# Autodesk Inventor assembly: 4thRhinoRobot
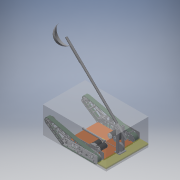
[picture p0: Inventor's stored thumbnail of the model, 180x180]
Saved by Autodesk Inventor 2016 SP1 (Build 200210100, 210)
## iProperties
Created: 2015-12-30
Part Number: 4thRhinoRobot
Document SubType Name: Assembly
Designer: steele
Mass: 23511.9 g
Surface Area: 38256.8 cm^2
Volume: 14882.3 cm^3
Density: 1.57986 g/cm^3
Author: steele
## Documents named in this file (15)
- C:\snobotics\CAD-Development\robSteele\SnoBotics2016\4thCutRhinoRobot\4thRhinoRobot.iam
- C:\snobotics\CAD-Development\robSteele\SnoBotics2016\RhinoTrackDrive\am-3322+RhinoTrackDriveModule.iam
- C:\snobotics\CAD-Development\robSteele\SnoBotics2016\FirstCutRhinoRobot\BasePlate.ipt
- C:\snobotics\CAD-Development\robSteele\SnoBotics2016\RhinoTrackDrive\am-3322+RhinoTrackDriveModule_MIR.iam
- C:\snobotics\autodesk\2015\FRC_KOP_2015\Motors\MOT_CIM-Motor_217-2000.iam
- C:\snobotics\CAD-Development\robSteele\SnoBotics2016\2ndCutAtCatapultRobot\catapultArmSupportStructure.ipt
- C:\snobotics\CAD-Development\robSteele\SnoBotics2016\FirstCutCatapult\CatapultAxel.ipt
- C:\snobotics\CAD-Development\robSteele\SnoBotics2016\2ndCutAtCatapultRobot\6498K330.ipt
- C:\snobotics\CAD-MfgResources\McMaster-Carr\Air Cylinder\Universal Mount\Single Acting Spring Return\3_4 bore 6 stroke\6498K045.ipt
- C:\snobotics\CAD-Development\robSteele\SnoBotics2016\FirstCutCatapult\cArmPully.ipt
- C:\snobotics\CAD-Development\robSteele\SnoBotics2016\3rdCutRhinoCatapultRobot\rearBox.ipt
- C:\snobotics\CAD-Development\robSteele\SnoBotics2016\3rdCutRhinoCatapultRobot\frontBox.ipt
- C:\snobotics\CAD-Development\robSteele\SnoBotics2016\FirstCutCatapult\roundCatapultArm.ipt
- C:\snobotics\CAD-Development\robSteele\SnoBotics2016\3rdCutRhinoCatapultRobot\rhinoRobotVolume.ipt
- C:\snobotics\CAD-Development\robSteele\SnoBotics2016\3rdCutRhinoCatapultRobot\oneHalfSaladBowl.ipt
## Components (18 placed, 14 different names)
1. am-3322+RhinoTrackDriveModule:1 [sub-assembly] — Flush:1, Mate:2, Flush:2, Flush:3, Insert:1, Insert:2, Flush:11
2. BasePlate:1 — Mate:2, Flush:2, Flush:3, Flush:4, Flush:5, Mate:3, Mate:4, Flush:6, Mate:7, Mate:8, Flush:7, Mate:10, Mate:11, Flush:8, Mate:12, Mate:13, Flush:9, Mate:14
3. am-3322+RhinoTrackDriveModule_MIR:1 [sub-assembly] — Mate:1, Flush:4, Flush:5, Insert:3, Insert:4
4. MOT_CIM-Motor_217-2000:1 [sub-assembly] — Insert:1
5. MOT_CIM-Motor_217-2000:2 [sub-assembly] — Insert:2
6. MOT_CIM-Motor_217-2000:3 [sub-assembly] — Insert:3
7. MOT_CIM-Motor_217-2000:4 [sub-assembly] — Insert:4
8. catapultArmSupportStructure:1 — Mate:3, Mate:4, Flush:6, Mate:6, Insert:5, Insert:6, Rotational:1
9. CatapultAxel:2 — Mate:6
10. 6498K330:1 — Mate:7, Mate:8, Flush:7, Mate:9
11. 6498K045:1 — Mate:9
12. cArmPully:1 — Insert:5
13. rearBox:1 — Mate:10, Mate:11, Flush:8, Flush:10
14. frontBox:1 — Mate:12, Mate:13, Flush:9
15. CatapultAxel:3 — Insert:6
16. roundCatapultArm:1 — Rotational:1, Flush:12, Mate:15
17. rhinoRobotVolume:1 — Mate:14, Flush:10, Flush:11
18. oneHalfSaladBowl:1 — Flush:12, Mate:15
## Relationships (33: Mate 14, Flush 12, Insert 6, RevoluteJoint 1)
- Flush:1 (254 mm): am-3322+RhinoTrackDriveModule:1
- Mate:1 (165.1 mm): am-3322+RhinoTrackDriveModule_MIR:1
- Mate:2: am-3322+RhinoTrackDriveModule:1 ↔ BasePlate:1
- Flush:2: am-3322+RhinoTrackDriveModule:1 ↔ BasePlate:1
- Flush:3: am-3322+RhinoTrackDriveModule:1 ↔ BasePlate:1
- Flush:4: BasePlate:1 ↔ am-3322+RhinoTrackDriveModule_MIR:1
- Flush:5: BasePlate:1 ↔ am-3322+RhinoTrackDriveModule_MIR:1
- Insert:1: am-3322+RhinoTrackDriveModule:1 ↔ MOT_CIM-Motor_217-2000:1
- Insert:2: am-3322+RhinoTrackDriveModule:1 ↔ MOT_CIM-Motor_217-2000:2
- Insert:3: am-3322+RhinoTrackDriveModule_MIR:1 ↔ MOT_CIM-Motor_217-2000:3
- Insert:4: am-3322+RhinoTrackDriveModule_MIR:1 ↔ MOT_CIM-Motor_217-2000:4
- Mate:3: BasePlate:1 ↔ catapultArmSupportStructure:1
- Mate:4: BasePlate:1 ↔ catapultArmSupportStructure:1
- Flush:6 (-63.5 mm): BasePlate:1 ↔ catapultArmSupportStructure:1
- Mate:6: catapultArmSupportStructure:1 ↔ CatapultAxel:2
- Mate:7: BasePlate:1 ↔ 6498K330:1
- Mate:8: BasePlate:1 ↔ 6498K330:1
- Flush:7 (279.4 mm): BasePlate:1 ↔ 6498K330:1
- Mate:9: 6498K330:1 ↔ 6498K045:1
- Insert:5 (12.7 mm): catapultArmSupportStructure:1 ↔ cArmPully:1
- Mate:10: BasePlate:1 ↔ rearBox:1
- Mate:11: BasePlate:1 ↔ rearBox:1
- Flush:8: BasePlate:1 ↔ rearBox:1
- Mate:12: BasePlate:1 ↔ frontBox:1
- Mate:13: BasePlate:1 ↔ frontBox:1
- Flush:9: BasePlate:1 ↔ frontBox:1
- Insert:6: catapultArmSupportStructure:1 ↔ CatapultAxel:3
- Rotational:1 [RevoluteJoint] (-12.7 mm): catapultArmSupportStructure:1 ↔ roundCatapultArm:1
- Mate:14: BasePlate:1 ↔ rhinoRobotVolume:1
- Flush:10: rearBox:1 ↔ rhinoRobotVolume:1
- Flush:11: am-3322+RhinoTrackDriveModule:1 ↔ rhinoRobotVolume:1
- Flush:12 (-12.7 mm): roundCatapultArm:1 ↔ oneHalfSaladBowl:1
- Mate:15: roundCatapultArm:1 ↔ oneHalfSaladBowl:1
## Named parameters: batteryWidth = 179.578 mm, centerOfBattery = 89.789 mm, widthOfRoboRIO = 146.1516 mm, centerOfRobotRIO = 73.0758 mm
